# Autodesk Inventor assembly: MG-Chip Kicker
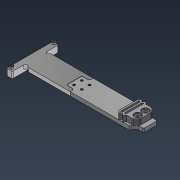
[picture p0: Inventor's stored thumbnail of the model, 180x180]
Saved by Autodesk Inventor 2022.1 (Build 261234020, 234B)
## iProperties
Part Number: MG-Chip Kicker
Material: Generisch
Document SubType Name: Assembly
Designer: rYan
Mass: 73.5332 g
Surface Area: 108.095 cm^2
Volume: 14.6899 cm^3
Density: 5.00571 g/cm^3
Author: rYan
## Documents named in this file (7)
- D:\TIGERsGIT\Hardware\mechanik\2020\Inventor\Robot\Kicker\MG-Chip Kicker.iam
- D:\TIGERsGIT\Hardware\mechanik\2020\Inventor\Robot\Kicker\Kicker Chip.ipt
- D:\TIGERsGIT\Hardware\mechanik\2020\Inventor\Robot\Kicker\Kicker Eisen.ipt
- D:\TIGERsGIT\Hardware\mechanik\2020\Inventor\Inhaltscenter\de-DE\ISO 4762(2)\ISO 4762 - M2 x 6ISO.ipt
- D:\TIGERsGIT\Hardware\mechanik\2020\Inventor\Robot\Kicker\Kickerdaempfer.ipt
- D:\TIGERsGIT\Hardware\mechanik\2020\Inventor\Inhaltscenter\de-DE\DIN 7984\DIN 7984 - M4 x 6.ipt
- D:\TIGERsGIT\Hardware\mechanik\2020\Inventor\Purchased Parts\ISO 10642 - M3 x 4.ipt
## Components (11 placed, 6 different names)
1. Kicker Chip:1 — Fluchtend:1, Fluchtend:2, Fluchtend:3, Einfügen:9, Einfügen:10, Einfügen:14, Passend:3, Einfügen:15, Einfügen:16, Einfügen:17, Einfügen:18
2. Kicker Eisen:1 — Einfügen:13, Passend:2, Einfügen:14, Passend:3
3. ISO 4762 M2 x 6:1 — Einfügen:10
4. ISO 4762 M2 x 6:2 — Einfügen:9
5. Kickerdaempfer:1 — Einfügen:13, Passend:2
6. DIN 7984 M4 x 6:1
7. DIN 7984 M4 x 6:2
8. ISO 10642 M3 x  6:1 — Einfügen:18
9. ISO 10642 M3 x  6:2 — Einfügen:17
10. ISO 10642 M3 x  6:3 — Einfügen:16
11. ISO 10642 M3 x  6:4 — Einfügen:15
## Relationships (15: Insert 10, Flush 3, Mate 2)
- Fluchtend:1 [Flush]: Kicker Chip:1
- Fluchtend:2 [Flush]: Kicker Chip:1
- Fluchtend:3 [Flush]: Kicker Chip:1
- Einfügen:9 [Insert] (1 mm): Kicker Chip:1 ↔ ISO 4762 M2 x 6:2
- Einfügen:10 [Insert] (1 mm): Kicker Chip:1 ↔ ISO 4762 M2 x 6:1
- [Insert]: Kickerdaempfer:1 ↔ DIN 7984 M4 x 6:2
- [Insert]: Kickerdaempfer:1 ↔ DIN 7984 M4 x 6:1
- Einfügen:13 [Insert]: Kicker Eisen:1 ↔ Kickerdaempfer:1
- Passend:2 [Mate]: Kicker Eisen:1 ↔ Kickerdaempfer:1
- Einfügen:14 [Insert]: Kicker Chip:1 ↔ Kicker Eisen:1
- Passend:3 [Mate]: Kicker Chip:1 ↔ Kicker Eisen:1
- Einfügen:15 [Insert]: Kicker Chip:1 ↔ ISO 10642 M3 x  6:4
- Einfügen:16 [Insert]: Kicker Chip:1 ↔ ISO 10642 M3 x  6:3
- Einfügen:17 [Insert]: Kicker Chip:1 ↔ ISO 10642 M3 x  6:2
- Einfügen:18 [Insert]: Kicker Chip:1 ↔ ISO 10642 M3 x  6:1
